# Autodesk Inventor assembly: Kitchen assy
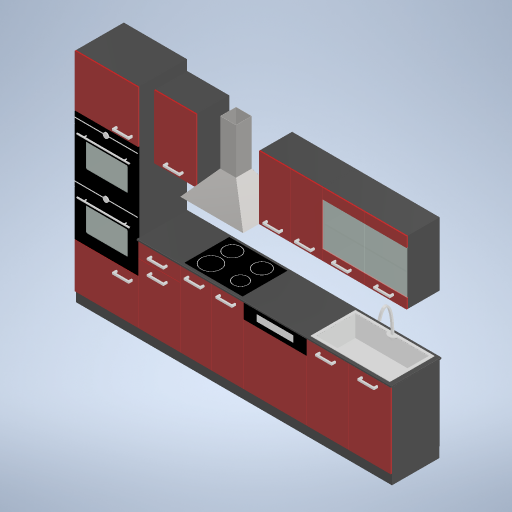
[picture p0: Inventor's stored thumbnail of the model, 512x512]
Saved by Autodesk Inventor 2024 (Build 280153000, 153)
## iProperties
Created: 2023-06-24
Part Number: Kitchen assy
Document SubType Name: Assembly
Designer: 69
Author: 69
## Documents named in this file (20)
- C:\Users\69\Desktop\git new\Kitchen\Kitchen assy.iam
- C:\Users\69\Desktop\git new\Kitchen\Base Cabinet 1\Base Cabinet 1 assy.iam
- C:\Users\69\Desktop\git new\Kitchen\Base Cabinet 2\Base Cabinet 2 assy.iam
- C:\Users\69\Desktop\git new\Kitchen\Base Cabinet 3\Base Cabinet 3 assy.iam
- C:\Users\69\Desktop\git new\Kitchen\Base Cabinet 4\Base Cabinet 4 assy.iam
- C:\Users\69\Desktop\git new\Kitchen\Sketch Geometry.ipt
- C:\Users\69\Desktop\git new\Kitchen\Wall Cabinet 1\Wall Cabinet 1 assy.iam
- C:\Users\69\Desktop\git new\Kitchen\Wall Cabinet 2\Wall Cabinet 2 assy.iam
- C:\Users\69\Desktop\git new\Kitchen\Wall Cabinet 3\Wall Cabinet 3 assy.iam
- C:\Users\69\Desktop\git new\Kitchen\Hood\Hood assy.iam
- C:\Users\69\Desktop\git new\Kitchen\Dishwasher Door\Dishwasher Door assy.iam
- C:\Users\69\Desktop\git new\Kitchen\Countertop\Countertop assy.iam
- C:\Users\69\Desktop\git new\Kitchen\Toe Kick\Toe Kick assy.iam
- C:\Users\69\Desktop\git new\Kitchen\Dummy Stove\Dummy Stove assy.iam
- C:\Users\69\Desktop\git new\Kitchen\Dummy Stove Plate\Dummy Stove Plate.iam
- C:\Users\69\Desktop\git new\Kitchen\Sink\Sink assy.iam
- C:\Users\69\Desktop\git new\Kitchen\Dummy Washing Machine\Dummy Washing Machine.iam
- C:\Users\69\Desktop\git new\Kitchen\Handle\Handle.iam
- C:\Users\69\Desktop\git new\Kitchen\Handle\Sketch Geometry 2.ipt
- C:\Users\69\Desktop\git new\Kitchen\Handle\Sketch Geometry 4.ipt
## Components (32 placed, 19 different names)
1. Sketch Geometry:1 — Mate:1, Mate:2, Mate:3, Mate:5, Mate:7, Mate:8, Mate:9, Mate:10, Mate:11, Mate:12, Mate:13, Mate:14, Mate:15, Mate:19
2. Base Cabinet 1 assy:1 [sub-assembly] — Mate:1, Mate:2, Mate:4, Mate:25, Mate:26, Mate:27, Mate:28, Flush:1, Flush:2
3. Base Cabinet 2 assy:1 [sub-assembly] — Mate:3, Mate:4, Mate:6, Mate:21, Mate:22
4. Base Cabinet 3 assy:1 [sub-assembly] — Mate:5, Mate:6, Mate:18, Mate:23
5. Base Cabinet 4 assy:1 [sub-assembly] — Mate:7, Mate:8, Mate:17, Mate:24, Mate:34
6. Wall Cabinet 1 assy:1 [sub-assembly] — Mate:9, Mate:10, Mate:20, Flush:3, Flush:4
7. Wall Cabinet 2 assy:1 [sub-assembly] — Mate:11, Mate:12, Mate:16
8. Wall Cabinet 3 assy:1 [sub-assembly] — Mate:13, Mate:14
9. Hood assy:1 [sub-assembly] — Mate:15, Mate:16, Mate:19, Mate:20
10. Dishwasher Door assy:1 [sub-assembly] — Mate:17, Mate:18, Mate:33
11. Countertop assy:1 [sub-assembly] — Mate:21, Mate:22, Mate:29, Mate:30, Mate:31, Mate:32
12. Toe Kick assy:1 [sub-assembly] — Mate:23, Mate:24
13. Dummy Stove assy:1 [sub-assembly] — Mate:26, Mate:28
14. Dummy Stove assy:2 [sub-assembly] — Mate:25, Mate:27
15. Dummy Stove Plate:1 [sub-assembly] — Mate:29, Mate:30
16. Sink assy:1 [sub-assembly] — Mate:31, Mate:32
17. Dummy Washing Machine:1 [sub-assembly] — Mate:33, Mate:34
18. Sketch Geometry 2 — Flush:1, Flush:2, Mate:35, Mate:36, Mate:37, Mate:38, Mate:39, Mate:40, Mate:41, Mate:42, Mate:43, Mate:44, Mate:45, Mate:46, Mate:47, Mate:48, Mate:49, Mate:50
19. Handle:1 [sub-assembly] — Mate:35, Mate:36
20. Handle:2 [sub-assembly] — Mate:37, Mate:38
21. Handle:3 [sub-assembly] — Mate:39, Mate:45
22. Handle:4 [sub-assembly] — Mate:42, Mate:48
23. Handle:5 [sub-assembly] — Mate:40, Mate:46
24. Handle:6 [sub-assembly] — Mate:41, Mate:47
25. Handle:7 [sub-assembly] — Mate:43, Mate:49
26. Handle:8 [sub-assembly] — Mate:44, Mate:50
27. Sketch Geometry 3 — Flush:3, Flush:4, Mate:51, Mate:52, Mate:53, Mate:54, Mate:55, Mate:56, Mate:57, Mate:58, Mate:59, Mate:60
28. Handle:9 [sub-assembly] — Mate:51, Mate:56
29. Handle:10 [sub-assembly] — Mate:53, Mate:58
30. Handle:11 [sub-assembly] — Mate:52, Mate:57
31. Handle:12 [sub-assembly] — Mate:55, Mate:60
32. Handle:13 [sub-assembly] — Mate:54, Mate:59
## Relationships (64: Mate 60, Flush 4)
- Mate:1: Sketch Geometry:1 ↔ Base Cabinet 1 assy:1
- Mate:2: Sketch Geometry:1 ↔ Base Cabinet 1 assy:1
- Mate:3: Sketch Geometry:1 ↔ Base Cabinet 2 assy:1
- Mate:4: Base Cabinet 1 assy:1 ↔ Base Cabinet 2 assy:1
- Mate:5: Sketch Geometry:1 ↔ Base Cabinet 3 assy:1
- Mate:6: Base Cabinet 2 assy:1 ↔ Base Cabinet 3 assy:1
- Mate:7: Sketch Geometry:1 ↔ Base Cabinet 4 assy:1
- Mate:8: Sketch Geometry:1 ↔ Base Cabinet 4 assy:1
- Mate:9: Sketch Geometry:1 ↔ Wall Cabinet 1 assy:1
- Mate:10: Sketch Geometry:1 ↔ Wall Cabinet 1 assy:1
- Mate:11: Sketch Geometry:1 ↔ Wall Cabinet 2 assy:1
- Mate:12: Sketch Geometry:1 ↔ Wall Cabinet 2 assy:1
- Mate:13: Sketch Geometry:1 ↔ Wall Cabinet 3 assy:1
- Mate:14: Sketch Geometry:1 ↔ Wall Cabinet 3 assy:1
- Mate:15: Sketch Geometry:1 ↔ Hood assy:1
- Mate:16: Wall Cabinet 2 assy:1 ↔ Hood assy:1
- Mate:17: Base Cabinet 4 assy:1 ↔ Dishwasher Door assy:1
- Mate:18: Base Cabinet 3 assy:1 ↔ Dishwasher Door assy:1
- Mate:19: Sketch Geometry:1 ↔ Hood assy:1
- Mate:20: Wall Cabinet 1 assy:1 ↔ Hood assy:1
- Mate:21: Base Cabinet 2 assy:1 ↔ Countertop assy:1
- Mate:22: Base Cabinet 2 assy:1 ↔ Countertop assy:1
- Mate:23: Base Cabinet 3 assy:1 ↔ Toe Kick assy:1
- Mate:24: Base Cabinet 4 assy:1 ↔ Toe Kick assy:1
- Mate:25: Base Cabinet 1 assy:1 ↔ Dummy Stove assy:2
- Mate:26: Base Cabinet 1 assy:1 ↔ Dummy Stove assy:1
- Mate:27 (3 mm): Base Cabinet 1 assy:1 ↔ Dummy Stove assy:2
- Mate:28 (3 mm): Base Cabinet 1 assy:1 ↔ Dummy Stove assy:1
- Mate:29: Countertop assy:1 ↔ Dummy Stove Plate:1
- Mate:30: Countertop assy:1 ↔ Dummy Stove Plate:1
- Mate:31: Countertop assy:1 ↔ Sink assy:1
- Mate:32: Countertop assy:1 ↔ Sink assy:1
- Mate:33: Dishwasher Door assy:1 ↔ Dummy Washing Machine:1
- Mate:34: Base Cabinet 4 assy:1 ↔ Dummy Washing Machine:1
- Flush:1: Base Cabinet 1 assy:1 ↔ Sketch Geometry 2
- Flush:2: Base Cabinet 1 assy:1 ↔ Sketch Geometry 2
- Mate:35: Sketch Geometry 2 ↔ Handle:1
- Mate:36: Sketch Geometry 2 ↔ Handle:1
- Mate:37: Sketch Geometry 2 ↔ Handle:2
- Mate:38: Sketch Geometry 2 ↔ Handle:2
- Mate:39: Sketch Geometry 2 ↔ Handle:3
- Mate:40: Sketch Geometry 2 ↔ Handle:5
- Mate:41: Sketch Geometry 2 ↔ Handle:6
- Mate:42: Sketch Geometry 2 ↔ Handle:4
- Mate:43: Sketch Geometry 2 ↔ Handle:7
- Mate:44: Sketch Geometry 2 ↔ Handle:8
- Mate:45: Sketch Geometry 2 ↔ Handle:3
- Mate:46: Sketch Geometry 2 ↔ Handle:5
- Mate:47: Sketch Geometry 2 ↔ Handle:6
- Mate:48: Sketch Geometry 2 ↔ Handle:4
- Mate:49: Sketch Geometry 2 ↔ Handle:7
- Mate:50: Sketch Geometry 2 ↔ Handle:8
- Flush:3: Wall Cabinet 1 assy:1 ↔ Sketch Geometry 3
- Flush:4: Wall Cabinet 1 assy:1 ↔ Sketch Geometry 3
- Mate:51: Sketch Geometry 3 ↔ Handle:9
- Mate:52: Sketch Geometry 3 ↔ Handle:11
- Mate:53: Sketch Geometry 3 ↔ Handle:10
- Mate:54: Sketch Geometry 3 ↔ Handle:13
- Mate:55: Sketch Geometry 3 ↔ Handle:12
- Mate:56: Sketch Geometry 3 ↔ Handle:9
- Mate:57: Sketch Geometry 3 ↔ Handle:11
- Mate:58: Sketch Geometry 3 ↔ Handle:10
- Mate:59: Sketch Geometry 3 ↔ Handle:13
- Mate:60: Sketch Geometry 3 ↔ Handle:12
